# Autodesk Inventor assembly: schnellwechsler
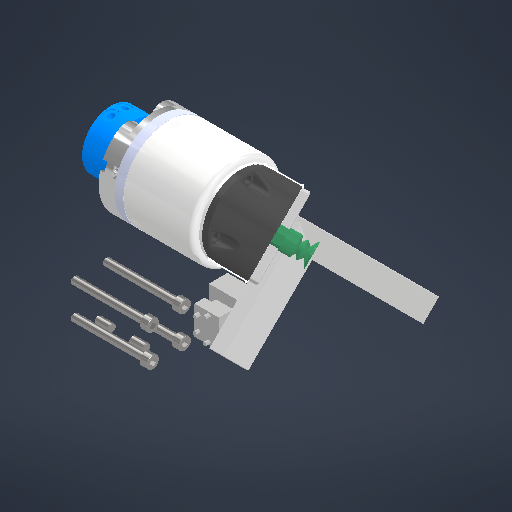
[picture p0: Inventor's stored thumbnail of the model, 512x512]
Saved by Autodesk Inventor 2026.1 (Build 301233020, 233B)
## iProperties
Created: 2025-11-06
Part Number: schnellwechsler
Document SubType Name: Assembly
Designer: neume
Sending System: Autodesk Inventor 2026
Preprocessor: ST-DEVELOPER v20.1
Title: schnellwechsler.stp
Author: peter
## Documents named in this file (9)
- C:\Users\neume\Desktop\MCI\Robotik_Labor\3D\schnellwechsler.iam
- C:\Users\neume\Desktop\MCI\Robotik_Projekt\Optimierung-Laboraufgabe-Robotik\Konstruktionen STEP\schnellwechsler\schnellwechsler\VerbindungselementRoboter.ipt
- C:\Users\neume\Desktop\MCI\Robotik_Projekt\Optimierung-Laboraufgabe-Robotik\Konstruktionen STEP\schnellwechsler\schnellwechsler\WER2000FSI32-05-B.ipt
- C:\Users\neume\Desktop\MCI\Robotik_Projekt\Optimierung-Laboraufgabe-Robotik\Konstruktionen STEP\schnellwechsler\schnellwechsler\HWR2000_Festteil_HWR2031F1.ipt
- C:\Users\neume\Desktop\MCI\Robotik_Projekt\Optimierung-Laboraufgabe-Robotik\Konstruktionen STEP\schnellwechsler\schnellwechsler\ISO 2338 - 5 h8 x 10.ipt
- C:\Users\neume\Desktop\MCI\Robotik_Projekt\Optimierung-Laboraufgabe-Robotik\Konstruktionen STEP\schnellwechsler\schnellwechsler\ISO 4762 - M5 x 50ISO.ipt
- C:\Users\neume\Desktop\MCI\Robotik_Projekt\Optimierung-Laboraufgabe-Robotik\Konstruktionen STEP\schnellwechsler\schnellwechsler\HWR2000_Losteil_HWR2031L1.ipt
- C:\Users\neume\Desktop\MCI\Robotik_Projekt\Optimierung-Laboraufgabe-Robotik\Konstruktionen STEP\schnellwechsler\schnellwechsler\WER2000LSI32-05.ipt
- C:\Users\neume\Desktop\MCI\Robotik_Labor\3D\endeffector.iam
## Components (12 placed, 8 different names)
1. endeffector:1 [sub-assembly] — Passend:1, Passend:2
2. VerbindungselementRoboter:1
3. WER2000FSI32-05-B:1
4. HWR2000_Festteil_HWR2031F1:1
5. ISO 2338 - 5 h8 x 10:1
6. ISO 4762 - M5 x 50ISO:1
7. ISO 4762 - M5 x 50ISO:2
8. ISO 4762 - M5 x 50ISO:3
9. ISO 4762 - M5 x 50ISO:4
10. ISO 2338 - 5 h8 x 10:2
11. HWR2000_Losteil_HWR2031L1:1 — Passend:1, Passend:2
12. WER2000LSI32-05:1
## Relationships (2: Mate 2)
- Passend:1 [Mate]: endeffector:1 ↔ HWR2000_Losteil_HWR2031L1:1
- Passend:2 [Mate]: endeffector:1 ↔ HWR2000_Losteil_HWR2031L1:1
